# Autodesk Inventor assembly: Assembly_Holder
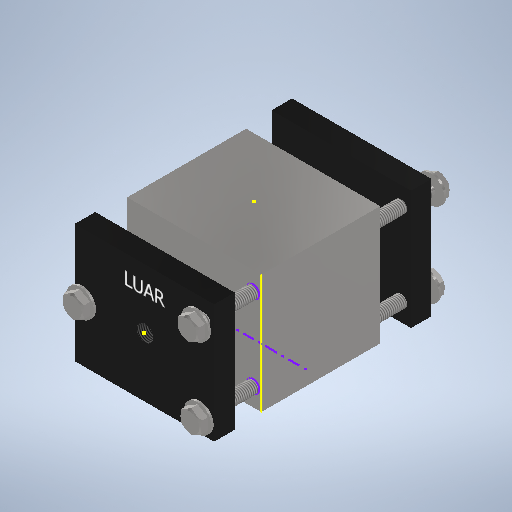
[picture p0: Inventor's stored thumbnail of the model, 512x512]
Saved by Autodesk Inventor 2025.1 (Build 291241000, 241)
## iProperties
Created: 2024-09-22
Part Number: Assembly_Holder
Document SubType Name: Assembly
Designer: JuhenFW
Author: JuhenFW
## Documents named in this file (5)
- D:\Proyek\Holder_Camera\Assembly_Holder.iam
- D:\Proyek\Holder_Camera\Camera.ipt
- D:\Proyek\Holder_Camera\Part2.ipt
- D:\Proyek\Holder_Camera\Part2_MIR2.ipt
- C:\Users\JuhenFW\Documents\Inventor\Content Center Files\R2025\en-US\AS 1427(00)\AS 1427 - M3 x 16(4).ipt
## Components (9 placed, 4 different names)
1. Camera:1 — Flush:2, Flush:4, Mate:1, Mate:2, Cylindrical:7, Cylindrical:8
2. Part2:1 — Flush:2, Mate:1, Cylindrical:1, Cylindrical:2, Cylindrical:3
3. Part2_MIR2:1 — Flush:4, Mate:2, Cylindrical:4, Cylindrical:5, Cylindrical:6
4. AS 1427 - Metric M3 x 16:1 — Cylindrical:1
5. AS 1427 - Metric M3 x 16:2 — Cylindrical:2, Cylindrical:7
6. AS 1427 - Metric M3 x 16:3 — Cylindrical:3
7. AS 1427 - Metric M3 x 16:4 — Cylindrical:4
8. AS 1427 - Metric M3 x 16:5 — Cylindrical:6
9. AS 1427 - Metric M3 x 16:6 — Cylindrical:5, Cylindrical:8
## Relationships (12: CylindricalJoint 8, Flush 2, Mate 2)
- Flush:2: Camera:1 ↔ Part2:1
- Flush:4: Camera:1 ↔ Part2_MIR2:1
- Mate:1 (7 mm): Camera:1 ↔ Part2:1
- Mate:2 (7 mm): Camera:1 ↔ Part2_MIR2:1
- Cylindrical:1: Part2:1 ↔ AS 1427 - Metric M3 x 16:1
- Cylindrical:2: Part2:1 ↔ AS 1427 - Metric M3 x 16:2
- Cylindrical:3: Part2:1 ↔ AS 1427 - Metric M3 x 16:3
- Cylindrical:4: Part2_MIR2:1 ↔ AS 1427 - Metric M3 x 16:4
- Cylindrical:5: Part2_MIR2:1 ↔ AS 1427 - Metric M3 x 16:6
- Cylindrical:6: Part2_MIR2:1 ↔ AS 1427 - Metric M3 x 16:5
- Cylindrical:7: Camera:1 ↔ AS 1427 - Metric M3 x 16:2
- Cylindrical:8: Camera:1 ↔ AS 1427 - Metric M3 x 16:6
